# Autodesk Inventor assembly: AssemblyFidget
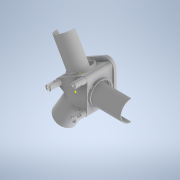
[picture p0: Inventor's stored thumbnail of the model, 180x180]
Saved by Autodesk Inventor 2022.4 (Build 264492010, 492A)
## iProperties
Created: 2023-09-20
Part Number: AssemblyFidget
Document SubType Name: Assembly
Designer: tmass
Author: tmass
## Documents named in this file (8)
- C:\Users\tmass\OneDrive\Bureau\UFO paper\3D models\Fidget\Inventor\AssemblyFidget.iam
- C:\Users\tmass\OneDrive\Bureau\UFO paper\3D models\Fidget\Inventor\Reactor small aircooled.ipt
- C:\Users\tmass\OneDrive\Bureau\UFO paper\3D models\Fidget\Inventor\Lid small.ipt
- C:\Users\tmass\OneDrive\Bureau\UFO paper\3D models\Fidget\Inventor\mini fidget foot.ipt
- C:\Users\tmass\OneDrive\Bureau\UFO paper\3D models\Fidget\Inventor\Coil holder.ipt
- C:\Users\tmass\OneDrive\Bureau\UFO paper\3D models\Fidget\Inventor\Kessil holder.ipt
- C:\Users\tmass\OneDrive\Bureau\UFO paper\3D models\Fidget\Inventor\Brass pillar.ipt
- C:\Users\tmass\OneDrive\Bureau\UFO paper\3D models\Fidget\Inventor\Plastic pillars.ipt
## Components (25 placed, 7 different names)
1. Reactor small aircooled:1 — Mate:1, Mate:2, Mate:3, Mate:4, Mate:5, Mate:6, Mate:7, Mate:8, Mate:9, Mate:10, Mate:11, Mate:12, Mate:13, Mate:14, Mate:15, Mate:16, Mate:17, Mate:18, Mate:19, Mate:20, Mate:21
2. Lid small:1 — Mate:4, Mate:5, Mate:6
3. mini fidget foot:1 — Mate:8, Mate:10
4. mini fidget foot:2 — Mate:7, Mate:11
5. mini fidget foot:3 — Mate:9, Mate:12
6. Coil holder:1 — Mate:1, Mate:2, Mate:3, Mate:22, Mate:23, Mate:24, Mate:25, Mate:26, Mate:27, Mate:28, Mate:29, Mate:30, Mate:31, Mate:32, Mate:33, Mate:34, Mate:35, Mate:36, Mate:37, Mate:38, Mate:39, Mate:40, Mate:41, Mate:42, Mate:43, Mate:44, Mate:45, Mate:46, Mate:47, Mate:48, Mate:49, Mate:50, Mate:51, Mate:52
7. Kessil holder:1 — Mate:13, Mate:14, Mate:15
8. Kessil holder:2 — Mate:16, Mate:17, Mate:18
9. Kessil holder:3 — Mate:19, Mate:20, Mate:21
10. Brass pillar:1 — Mate:25, Mate:27, Mate:53, Mate:54
11. Brass pillar:2 — Mate:23, Mate:26
12. Brass pillar:3 — Mate:24, Mate:28, Mate:55
13. Plastic pillars:1 — Mate:39, Mate:40
14. Plastic pillars:2 — Mate:47, Mate:48
15. Plastic pillars:3 — Mate:51, Mate:52
16. Plastic pillars:4 — Mate:45, Mate:46
17. Plastic pillars:5 — Mate:43, Mate:44
18. Plastic pillars:6 — Mate:41, Mate:42
19. Plastic pillars:7 — Mate:35, Mate:36
20. Plastic pillars:8 — Mate:31, Mate:32
21. Plastic pillars:9 — Mate:33, Mate:34
22. Plastic pillars:10 — Mate:37, Mate:38
23. Plastic pillars:11 — Mate:29, Mate:30
24. Plastic pillars:12 — Mate:49, Mate:50
25. Coil holder:2 — Mate:53, Mate:54, Mate:55
## Relationships (56: Mate 55, Angle 1)
- Mate:1: Reactor small aircooled:1 ↔ Coil holder:1
- Mate:2: Reactor small aircooled:1 ↔ Coil holder:1
- Mate:3 (1 mm): Reactor small aircooled:1 ↔ Coil holder:1
- Mate:4: Reactor small aircooled:1 ↔ Lid small:1
- Mate:5: Reactor small aircooled:1 ↔ Lid small:1
- Mate:6: Reactor small aircooled:1 ↔ Lid small:1
- Mate:7: Reactor small aircooled:1 ↔ mini fidget foot:2
- Mate:8: Reactor small aircooled:1 ↔ mini fidget foot:1
- Mate:9: Reactor small aircooled:1 ↔ mini fidget foot:3
- Mate:10: Reactor small aircooled:1 ↔ mini fidget foot:1
- Mate:11: Reactor small aircooled:1 ↔ mini fidget foot:2
- Mate:12: Reactor small aircooled:1 ↔ mini fidget foot:3
- Mate:13: Reactor small aircooled:1 ↔ Kessil holder:1
- Mate:14: Reactor small aircooled:1 ↔ Kessil holder:1
- Mate:15: Reactor small aircooled:1 ↔ Kessil holder:1
- Mate:16: Reactor small aircooled:1 ↔ Kessil holder:2
- Mate:17: Reactor small aircooled:1 ↔ Kessil holder:2
- Mate:18: Reactor small aircooled:1 ↔ Kessil holder:2
- Mate:19: Reactor small aircooled:1 ↔ Kessil holder:3
- Mate:20: Reactor small aircooled:1 ↔ Kessil holder:3
- Mate:21: Reactor small aircooled:1 ↔ Kessil holder:3
- Mate:22: Coil holder:1
- Angle:1 (0 deg)
- Mate:23: Coil holder:1 ↔ Brass pillar:2
- Mate:24: Coil holder:1 ↔ Brass pillar:3
- Mate:25: Coil holder:1 ↔ Brass pillar:1
- Mate:26: Coil holder:1 ↔ Brass pillar:2
- Mate:27: Coil holder:1 ↔ Brass pillar:1
- Mate:28: Coil holder:1 ↔ Brass pillar:3
- Mate:29: Coil holder:1 ↔ Plastic pillars:11
- Mate:30: Coil holder:1 ↔ Plastic pillars:11
- Mate:31: Coil holder:1 ↔ Plastic pillars:8
- Mate:32: Coil holder:1 ↔ Plastic pillars:8
- Mate:33: Coil holder:1 ↔ Plastic pillars:9
- Mate:34: Coil holder:1 ↔ Plastic pillars:9
- Mate:35: Coil holder:1 ↔ Plastic pillars:7
- Mate:36: Coil holder:1 ↔ Plastic pillars:7
- Mate:37: Coil holder:1 ↔ Plastic pillars:10
- Mate:38: Coil holder:1 ↔ Plastic pillars:10
- Mate:39: Coil holder:1 ↔ Plastic pillars:1
- Mate:40: Coil holder:1 ↔ Plastic pillars:1
- Mate:41: Coil holder:1 ↔ Plastic pillars:6
- Mate:42: Coil holder:1 ↔ Plastic pillars:6
- Mate:43: Coil holder:1 ↔ Plastic pillars:5
- Mate:44: Coil holder:1 ↔ Plastic pillars:5
- Mate:45: Coil holder:1 ↔ Plastic pillars:4
- Mate:46: Coil holder:1 ↔ Plastic pillars:4
- Mate:47: Coil holder:1 ↔ Plastic pillars:2
- Mate:48: Coil holder:1 ↔ Plastic pillars:2
- Mate:49: Coil holder:1 ↔ Plastic pillars:12
- Mate:50: Coil holder:1 ↔ Plastic pillars:12
- Mate:51: Coil holder:1 ↔ Plastic pillars:3
- Mate:52: Coil holder:1 ↔ Plastic pillars:3
- Mate:53: Brass pillar:1 ↔ Coil holder:2
- Mate:54: Brass pillar:1 ↔ Coil holder:2
- Mate:55: Brass pillar:3 ↔ Coil holder:2
